# Autodesk Inventor assembly: pulleyBracketAssembly
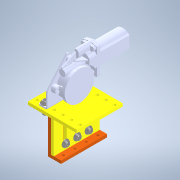
[picture p0: Inventor's stored thumbnail of the model, 180x180]
Saved by Autodesk Inventor 2022.1 (Build 261234020, 234B)
## iProperties
Created: 2021-11-11
Part Number: pulleyBracketAssembly
Document SubType Name: Assembly
Designer: robst
Author: robst
## Documents named in this file (9)
- C:\git\CAD-Development\robSteele\pulleyBracketAssembly.iam
- C:\git\CAD-Development\robSteele\pullyBracketLowerPortion.ipt
- C:\git\CAD-Development\robSteele\pullyBracketTopPortion.ipt
- C:\git\CAD-Development\robSteele\snowBlowerAndMount.iam
- C:\Users\robst\Documents\Inventor\Content Center Files\R2021\en-US\ANSI B18.22.1\ANSI B18.22.1 - 1_4 - narrow - Type A.ipt
- C:\Users\robst\Documents\Inventor\Content Center Files\R2021\en-US\ANSI B18.21.1\ANSI B18.21.1 - 0.25.ipt
- C:\Users\robst\Documents\Inventor\Content Center Files\R2021\en-US\U UNC 2605\Unbrako - 1_4 x 1 - 20(10).ipt
- C:\Users\robst\Documents\Inventor\Content Center Files\R2021\en-US\IFI 100 107(2)\IFI 100_107 - 1_4 - 20 Metal Type.ipt
- C:\Users\robst\Documents\Inventor\Content Center Files\R2021\en-US\U UNC 2605\Unbrako - 1_4 x 1.1_4 - 20(10).ipt
## Components (33 placed, 8 different names)
1. pullyBracketLowerPortion:1 — Mate:1, Flush:1, Mate:2, Mate:18, Mate:20, Mate:22
2. pullyBracketTopPortion:1 — Mate:1, Flush:1, Mate:2, Insert:1, Insert:2, Mate:8, Mate:10, Mate:11, Mate:12, Mate:13, Mate:14, Mate:15, Mate:16, Mate:17, Mate:19, Mate:21
3. snowBlowerAndMount:1 [sub-assembly] — Insert:1, Insert:2, Mate:3, Mate:4, Mate:5, Mate:6, Mate:7, Mate:9
4. Plain Washer (Inch) 1/4 - narrow - Type A:1 — Mate:3, Mate:4, Insert:3
5. Helical Spring Lock Washers 0.25:1 — Insert:3, Insert:5
6. Unbrako UNC Hex Socket Button Cap - Inch 1/4 x 1:1 — Insert:5
7. Plain Washer (Inch) 1/4 - narrow - Type A:2 — Mate:7, Mate:8, Insert:7
8. Helical Spring Lock Washers 0.25:2 — Insert:7, Insert:9
9. Prevailing Torque Type Hex Nut - Inch (IFI) 1/4 - 20 Metal Type:1 — Insert:9
10. Plain Washer (Inch) 1/4 - narrow - Type A:3 — Mate:5, Mate:6, Insert:4
11. Helical Spring Lock Washers 0.25:3 — Insert:4, Insert:6
12. Unbrako UNC Hex Socket Button Cap - Inch 1/4 x 1:2 — Insert:6
13. Plain Washer (Inch) 1/4 - narrow - Type A:4 — Mate:9, Mate:10, Insert:8
14. Helical Spring Lock Washers 0.25:4 — Insert:8, Insert:10
15. Prevailing Torque Type Hex Nut - Inch (IFI) 1/4 - 20 Metal Type:2 — Insert:10
16. Plain Washer (Inch) 1/4 - narrow - Type A:5 — Mate:11, Mate:12, Insert:11
17. Helical Spring Lock Washers 0.25:5 — Insert:11, Insert:14
18. Unbrako UNC Hex Socket Button Cap - Inch 1/4 x 1.1/4:1 — Insert:14
19. Plain Washer (Inch) 1/4 - narrow - Type A:6 — Mate:17, Mate:18, Insert:17
20. Helical Spring Lock Washers 0.25:6 — Insert:17, Insert:20
21. Prevailing Torque Type Hex Nut - Inch (IFI) 1/4 - 20 Metal Type:3 — Insert:20
22. Plain Washer (Inch) 1/4 - narrow - Type A:7 — Mate:13, Mate:14, Insert:12
23. Plain Washer (Inch) 1/4 - narrow - Type A:8 — Mate:15, Mate:16, Insert:13
24. Helical Spring Lock Washers 0.25:7 — Insert:12, Insert:15
25. Helical Spring Lock Washers 0.25:8 — Insert:13, Insert:16
26. Unbrako UNC Hex Socket Button Cap - Inch 1/4 x 1.1/4:2 — Insert:15
27. Unbrako UNC Hex Socket Button Cap - Inch 1/4 x 1.1/4:3 — Insert:16
28. Plain Washer (Inch) 1/4 - narrow - Type A:9 — Mate:19, Mate:20, Insert:18
29. Plain Washer (Inch) 1/4 - narrow - Type A:10 — Mate:21, Mate:22, Insert:19
30. Helical Spring Lock Washers 0.25:9 — Insert:18, Insert:21
31. Helical Spring Lock Washers 0.25:10 — Insert:19, Insert:22
32. Prevailing Torque Type Hex Nut - Inch (IFI) 1/4 - 20 Metal Type:4 — Insert:21
33. Prevailing Torque Type Hex Nut - Inch (IFI) 1/4 - 20 Metal Type:5 — Insert:22
## Relationships (45: Mate 22, Insert 22, Flush 1)
- Mate:1: pullyBracketLowerPortion:1 ↔ pullyBracketTopPortion:1
- Flush:1: pullyBracketLowerPortion:1 ↔ pullyBracketTopPortion:1
- Mate:2: pullyBracketLowerPortion:1 ↔ pullyBracketTopPortion:1
- Insert:1: pullyBracketTopPortion:1 ↔ snowBlowerAndMount:1
- Insert:2: pullyBracketTopPortion:1 ↔ snowBlowerAndMount:1
- Mate:3: snowBlowerAndMount:1 ↔ Plain Washer (Inch) 1/4 - narrow - Type A:1
- Mate:4: snowBlowerAndMount:1 ↔ Plain Washer (Inch) 1/4 - narrow - Type A:1
- Mate:5: snowBlowerAndMount:1 ↔ Plain Washer (Inch) 1/4 - narrow - Type A:3
- Mate:6: snowBlowerAndMount:1 ↔ Plain Washer (Inch) 1/4 - narrow - Type A:3
- Insert:3: Plain Washer (Inch) 1/4 - narrow - Type A:1 ↔ Helical Spring Lock Washers 0.25:1
- Insert:4: Plain Washer (Inch) 1/4 - narrow - Type A:3 ↔ Helical Spring Lock Washers 0.25:3
- Insert:5: Helical Spring Lock Washers 0.25:1 ↔ Unbrako UNC Hex Socket Button Cap - Inch 1/4 x 1:1
- Insert:6: Helical Spring Lock Washers 0.25:3 ↔ Unbrako UNC Hex Socket Button Cap - Inch 1/4 x 1:2
- Mate:7: snowBlowerAndMount:1 ↔ Plain Washer (Inch) 1/4 - narrow - Type A:2
- Mate:8: pullyBracketTopPortion:1 ↔ Plain Washer (Inch) 1/4 - narrow - Type A:2
- Mate:9: snowBlowerAndMount:1 ↔ Plain Washer (Inch) 1/4 - narrow - Type A:4
- Mate:10: pullyBracketTopPortion:1 ↔ Plain Washer (Inch) 1/4 - narrow - Type A:4
- Insert:7: Plain Washer (Inch) 1/4 - narrow - Type A:2 ↔ Helical Spring Lock Washers 0.25:2
- Insert:8: Plain Washer (Inch) 1/4 - narrow - Type A:4 ↔ Helical Spring Lock Washers 0.25:4
- Insert:9: Helical Spring Lock Washers 0.25:2 ↔ Prevailing Torque Type Hex Nut - Inch (IFI) 1/4 - 20 Metal Type:1
- Insert:10: Helical Spring Lock Washers 0.25:4 ↔ Prevailing Torque Type Hex Nut - Inch (IFI) 1/4 - 20 Metal Type:2
- Mate:11: pullyBracketTopPortion:1 ↔ Plain Washer (Inch) 1/4 - narrow - Type A:5
- Mate:12: pullyBracketTopPortion:1 ↔ Plain Washer (Inch) 1/4 - narrow - Type A:5
- Mate:13: pullyBracketTopPortion:1 ↔ Plain Washer (Inch) 1/4 - narrow - Type A:7
- Mate:14: pullyBracketTopPortion:1 ↔ Plain Washer (Inch) 1/4 - narrow - Type A:7
- Mate:15: pullyBracketTopPortion:1 ↔ Plain Washer (Inch) 1/4 - narrow - Type A:8
- Mate:16: pullyBracketTopPortion:1 ↔ Plain Washer (Inch) 1/4 - narrow - Type A:8
- Insert:11: Plain Washer (Inch) 1/4 - narrow - Type A:5 ↔ Helical Spring Lock Washers 0.25:5
- Insert:12: Plain Washer (Inch) 1/4 - narrow - Type A:7 ↔ Helical Spring Lock Washers 0.25:7
- Insert:13: Plain Washer (Inch) 1/4 - narrow - Type A:8 ↔ Helical Spring Lock Washers 0.25:8
- Insert:14: Helical Spring Lock Washers 0.25:5 ↔ Unbrako UNC Hex Socket Button Cap - Inch 1/4 x 1.1/4:1
- Insert:15: Helical Spring Lock Washers 0.25:7 ↔ Unbrako UNC Hex Socket Button Cap - Inch 1/4 x 1.1/4:2
- Insert:16: Helical Spring Lock Washers 0.25:8 ↔ Unbrako UNC Hex Socket Button Cap - Inch 1/4 x 1.1/4:3
- Mate:17: pullyBracketTopPortion:1 ↔ Plain Washer (Inch) 1/4 - narrow - Type A:6
- Mate:18: pullyBracketLowerPortion:1 ↔ Plain Washer (Inch) 1/4 - narrow - Type A:6
- Mate:19: pullyBracketTopPortion:1 ↔ Plain Washer (Inch) 1/4 - narrow - Type A:9
- Mate:20: pullyBracketLowerPortion:1 ↔ Plain Washer (Inch) 1/4 - narrow - Type A:9
- Mate:21: pullyBracketTopPortion:1 ↔ Plain Washer (Inch) 1/4 - narrow - Type A:10
- Mate:22: pullyBracketLowerPortion:1 ↔ Plain Washer (Inch) 1/4 - narrow - Type A:10
- Insert:17: Plain Washer (Inch) 1/4 - narrow - Type A:6 ↔ Helical Spring Lock Washers 0.25:6
- Insert:18: Plain Washer (Inch) 1/4 - narrow - Type A:9 ↔ Helical Spring Lock Washers 0.25:9
- Insert:19: Plain Washer (Inch) 1/4 - narrow - Type A:10 ↔ Helical Spring Lock Washers 0.25:10
- Insert:20: Helical Spring Lock Washers 0.25:6 ↔ Prevailing Torque Type Hex Nut - Inch (IFI) 1/4 - 20 Metal Type:3
- Insert:21: Helical Spring Lock Washers 0.25:9 ↔ Prevailing Torque Type Hex Nut - Inch (IFI) 1/4 - 20 Metal Type:4
- Insert:22: Helical Spring Lock Washers 0.25:10 ↔ Prevailing Torque Type Hex Nut - Inch (IFI) 1/4 - 20 Metal Type:5
